# Autodesk Inventor assembly: 6 Omni Wheel
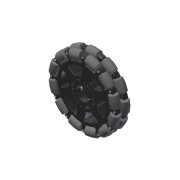
[picture p0: Inventor's stored thumbnail of the model, 180x180]
Saved by Autodesk Inventor 2013 (Build 170138000, 138)
## iProperties
Created: 2012-12-08
Part Number: 6 Omni Wheel
Document SubType Name: Assembly
Designer: niemitalo_dan
Translation Standard: STEP AP203
FileName: 217-2585.20121203.STEP
PreProcessor: SolidWorks 2012
PostProcessor: Build: 138, Release: 2013 RTM - Date: Thu 03/01/2012
Sent Units: inch
Uncertainty: 1e-05
Author: niemitalo_dan
## Documents named in this file (6)
- H:\Nemo\Documents\Robotics\VexPro\Omni Wheel\6 Omni Wheel.iam
- H:\Nemo\Documents\Robotics\VexPro\Omni Wheel\Components\Omni Wheel Inside 6 in.ipt
- H:\Nemo\Documents\Robotics\VexPro\Omni Wheel\Components\Omni Wheel Hub 6 inch.ipt
- H:\Nemo\Documents\Robotics\VexPro\Omni Wheel\Components\Omni Wheel Screw for VexPro.ipt
- H:\Nemo\Documents\Robotics\VexPro\Fasteners\Hex Standoff 8-32 x750.ipt
- H:\Nemo\Documents\Robotics\VexPro\Omni Wheel\Components\Omni Roller 6 in.iam
## Components (57 placed, 5 different names)
1. Omni Wheel Inside 6 in:1 — Mate:1, Mate:2, Angle:2, Mate:3, Mate:4, Mate:5, Mate:7, Mate:8, Mate:9, Mate:11
2. Omni Wheel Hub 6 inch:1 — Mate:6, Mate:7, Mate:8, Insert:3, Mate:10
3. Omni Wheel Hub 6 inch:2 — Angle:1, Insert:1, Mate:3, Mate:4, Mate:5, Insert:2, Mate:6, Mate:12
4. Hex Standoff 8-32 x750:1 — Angle:1, Insert:1
5. Hex Standoff 8-32 x750:2
6. Hex Standoff 8-32 x750:3
7. Hex Standoff 8-32 x750:4
8. Hex Standoff 8-32 x750:5
9. Hex Standoff 8-32 x750:6
10. Omni Roller 6 in:1 [sub-assembly] — Mate:9, Mate:10
11. Omni Roller 6 in:2 [sub-assembly] — Mate:11, Mate:12
12. Omni Wheel Screw for VexPro:16 — Insert:3
13. Omni Wheel Screw for VexPro:6 — Insert:2
14. Omni Roller 6 in:3 [sub-assembly]
15. Omni Roller 6 in:4 [sub-assembly]
16. Omni Wheel Screw for VexPro:17
17. Omni Wheel Screw for VexPro:18
18. Omni Roller 6 in:5 [sub-assembly]
19. Omni Roller 6 in:6 [sub-assembly]
20. Omni Wheel Screw for VexPro:19
21. Omni Wheel Screw for VexPro:20
22. Omni Roller 6 in:7 [sub-assembly]
23. Omni Roller 6 in:8 [sub-assembly]
24. Omni Wheel Screw for VexPro:21
25. Omni Wheel Screw for VexPro:22
26. Omni Roller 6 in:9 [sub-assembly]
27. Omni Roller 6 in:10 [sub-assembly]
28. Omni Wheel Screw for VexPro:23
29. Omni Wheel Screw for VexPro:24
30. Omni Roller 6 in:11 [sub-assembly]
31. Omni Roller 6 in:12 [sub-assembly]
32. Omni Wheel Screw for VexPro:25
33. Omni Wheel Screw for VexPro:26
34. Omni Roller 6 in:13 [sub-assembly]
35. Omni Roller 6 in:14 [sub-assembly]
36. Omni Wheel Screw for VexPro:27
37. Omni Wheel Screw for VexPro:28
38. Omni Roller 6 in:15 [sub-assembly]
39. Omni Roller 6 in:16 [sub-assembly]
40. Omni Wheel Screw for VexPro:29
41. Omni Wheel Screw for VexPro:30
42. Omni Roller 6 in:17 [sub-assembly]
43. Omni Roller 6 in:18 [sub-assembly]
44. Omni Wheel Screw for VexPro:31
45. Omni Wheel Screw for VexPro:32
46. Omni Roller 6 in:19 [sub-assembly]
47. Omni Roller 6 in:20 [sub-assembly]
48. Omni Wheel Screw for VexPro:33
49. Omni Wheel Screw for VexPro:34
50. Omni Roller 6 in:21 [sub-assembly]
51. Omni Roller 6 in:22 [sub-assembly]
52. Omni Wheel Screw for VexPro:35
53. Omni Wheel Screw for VexPro:36
54. Omni Roller 6 in:23 [sub-assembly]
55. Omni Roller 6 in:24 [sub-assembly]
56. Omni Wheel Screw for VexPro:37
57. Omni Wheel Screw for VexPro:38
## Component patterns: (6 elements, first: Hex Standoff 8-32 x750:1), (12 elements, first: Omni Roller 6 in:1 + Omni Roller 6 in:2 + Omni Wheel Screw for VexPro:16 + Omni Wheel Screw for VexPro:6)
## Relationships (17: Mate 12, Insert 3, Angle 2)
- Angle:1 (0 deg): Omni Wheel Hub 6 inch:2 ↔ Hex Standoff 8-32 x750:1
- Insert:1: Omni Wheel Hub 6 inch:2 ↔ Hex Standoff 8-32 x750:1
- Mate:1: Omni Wheel Inside 6 in:1
- Mate:2: Omni Wheel Inside 6 in:1
- Angle:2 (0 deg): Omni Wheel Inside 6 in:1
- Mate:3: Omni Wheel Inside 6 in:1 ↔ Omni Wheel Hub 6 inch:2
- Mate:4: Omni Wheel Inside 6 in:1 ↔ Omni Wheel Hub 6 inch:2
- Mate:5: Omni Wheel Inside 6 in:1 ↔ Omni Wheel Hub 6 inch:2
- Insert:2: Omni Wheel Hub 6 inch:2 ↔ Omni Wheel Screw for VexPro:6
- Mate:6: Omni Wheel Hub 6 inch:1 ↔ Omni Wheel Hub 6 inch:2
- Mate:7: Omni Wheel Inside 6 in:1 ↔ Omni Wheel Hub 6 inch:1
- Mate:8: Omni Wheel Inside 6 in:1 ↔ Omni Wheel Hub 6 inch:1
- Insert:3: Omni Wheel Hub 6 inch:1 ↔ Omni Wheel Screw for VexPro:16
- Mate:9: Omni Wheel Inside 6 in:1 ↔ Omni Roller 6 in:1
- Mate:10 (0.2413 mm): Omni Wheel Hub 6 inch:1 ↔ Omni Roller 6 in:1
- Mate:11: Omni Wheel Inside 6 in:1 ↔ Omni Roller 6 in:2
- Mate:12 (0.2413 mm): Omni Wheel Hub 6 inch:2 ↔ Omni Roller 6 in:2
